# Autodesk Inventor assembly: Pier
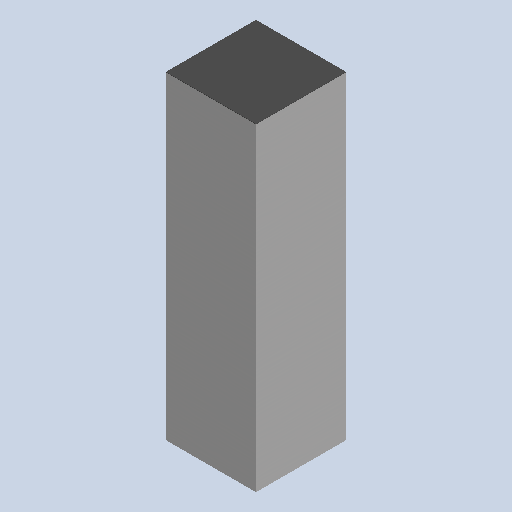
[picture p0: Inventor's stored thumbnail of the model, 512x512]
Saved by Autodesk Inventor 2025 (Build 290162010, 162A)
## iProperties
Created: 2024-09-15
Part Number: Pier
Document SubType Name: Assembly
Designer: Tom
Author: Tom
## Documents named in this file (3)
- C:\Users\Tom\Documents\Inventor\Mobility\Additional_Building\Pier.iam
- C:\Users\Tom\Documents\Inventor\Mobility\Additional_Building\Pier.ipt
- C:\Users\Tom\Documents\Inventor\Mobility\Additional_Building\Underlayment_For_Pier.ipt
## Components (2 placed, 2 different names)
1. Pier:1 — Mate:1, Flush:1, Flush:2, Mate:2, Flush:3, Mate:3
2. Underlayment_For_Pier:1 — Mate:1, Flush:1, Flush:2
## Relationships (6: Mate 3, Flush 3)
- Mate:1: Pier:1 ↔ Underlayment_For_Pier:1
- Flush:1: Pier:1 ↔ Underlayment_For_Pier:1
- Flush:2: Pier:1 ↔ Underlayment_For_Pier:1
- Mate:2: Pier:1
- Flush:3: Pier:1
- Mate:3: Pier:1
